# Autodesk Inventor assembly: Solid Curve 3D Print v25
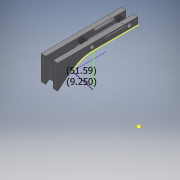
[picture p0: Inventor's stored thumbnail of the model, 180x180]
Saved by Autodesk Inventor 2018 (Build 220112000, 112)
## iProperties
Created: 2020-01-29
Part Number: Solid Curve 3D Print v25
Document SubType Name: Assembly
Designer: s-2512711
Author: s-2512711
## Documents named in this file (5)
- C:\Users\Weeb No1\Documents\GitHub\2020CAD\Gabriel Inventor Files (Shooter, Drivebase)\3D Printed Curve Assembly\Main Assembly\Solid Curve 3D Print v25.iam
- C:\Users\Weeb No1\Documents\GitHub\2020CAD\Gabriel Inventor Files (Shooter, Drivebase)\3D Printed Curve Assembly\Part Files\Polycord Roller WCP-0097 Rev1 v1.ipt
- C:\Users\Weeb No1\Documents\GitHub\2020CAD\Gabriel Inventor Files (Shooter, Drivebase)\3D Printed Curve Assembly\Part Files\RIGHT Bottom Part 1.ipt
- C:\Users\Weeb No1\Documents\GitHub\2020CAD\Gabriel Inventor Files (Shooter, Drivebase)\3D Printed Curve Assembly\Part Files\LEFT Bottom Part 1.ipt
- C:\Users\Weeb No1\Documents\GitHub\2020CAD\Gabriel Inventor Files (Shooter, Drivebase)\3D Printed Curve Assembly\Part Files\1x2 5in 1_16_ Beam v1.ipt
## Components (7 placed, 4 different names)
1. Polycord Roller WCP-0097 Rev1 v1:1 — Mate:3
2. Polycord Roller WCP-0097 Rev1 v1:2 — Mate:6
3. RIGHT Bottom Part 1:1 — Mate:1, Flush:1, Flush:2, Mate:3, Mate:5
4. LEFT Bottom Part 1:1 — Mate:4, Mate:6, Mate:7, Flush:3, Flush:4
5. Polycord Roller WCP-0097 Rev1 v1:3 — Mate:4
6. Polycord Roller WCP-0097 Rev1 v1:4 — Mate:5
7. 1x2 5in 1/16" Beam v1:2 — Mate:1, Flush:1, Flush:2, Mate:7, Flush:3, Flush:4
## Relationships (10: Mate 6, Flush 4)
- Mate:1: RIGHT Bottom Part 1:1 ↔ 1x2 5in 1/16" Beam v1:2
- Flush:1: RIGHT Bottom Part 1:1 ↔ 1x2 5in 1/16" Beam v1:2
- Flush:2: RIGHT Bottom Part 1:1 ↔ 1x2 5in 1/16" Beam v1:2
- Mate:3: Polycord Roller WCP-0097 Rev1 v1:1 ↔ RIGHT Bottom Part 1:1
- Mate:4: LEFT Bottom Part 1:1 ↔ Polycord Roller WCP-0097 Rev1 v1:3
- Mate:5: RIGHT Bottom Part 1:1 ↔ Polycord Roller WCP-0097 Rev1 v1:4
- Mate:6: Polycord Roller WCP-0097 Rev1 v1:2 ↔ LEFT Bottom Part 1:1
- Mate:7: LEFT Bottom Part 1:1 ↔ 1x2 5in 1/16" Beam v1:2
- Flush:3: LEFT Bottom Part 1:1 ↔ 1x2 5in 1/16" Beam v1:2
- Flush:4: LEFT Bottom Part 1:1 ↔ 1x2 5in 1/16" Beam v1:2
